# Autodesk Inventor assembly: Shooting Mechanism Assembly
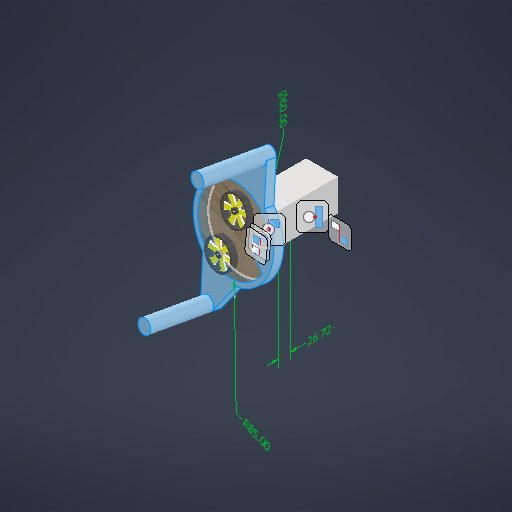
[picture p0: Inventor's stored thumbnail of the model, 512x512]
Saved by Autodesk Inventor 2026.2 (Build 302298000, 298)
## iProperties
Created: 2026-03-02
Part Number: Shooting Mechanism Assembly
Document SubType Name: Assembly
Designer: abdul
Author: abdul
## Documents named in this file (7)
- C:\Users\danda\OneDrive\Desktop\Basics Of Mecha\Project\Shooting Mechanism CAD\Shooting Mechanism Assembly.iam
- C:\Users\danda\OneDrive\Desktop\Basics Of Mecha\Project\Shooting Mechanism CAD\Base.ipt
- C:\Users\danda\OneDrive\Desktop\Basics Of Mecha\Project\Shooting Mechanism CAD\flywheel.ipt
- C:\Users\danda\OneDrive\Desktop\Basics Of Mecha\Project\Shooting Mechanism CAD\Dc Motor 3mm D Shaft.ipt
- C:\Users\danda\OneDrive\Desktop\Basics Of Mecha\Project\Ball Joint.iam
- C:\Users\danda\OneDrive\Desktop\Basics Of Mecha\Project\shootingstand.ipt
- C:\Users\danda\OneDrive\Desktop\Basics Of Mecha\Project\shooter handle.ipt
## Components (8 placed, 6 different names)
1. Base:1 — Mate:1, Mate:2, Mate:3, Mate:4, Mate:16, Mate:17, Flush:1, Mate:19, Mate:20
2. Dc Motor 3mm D Shaft:1 — Mate:1, Mate:4, Mate:9, Mate:11
3. Dc Motor 3mm D Shaft:2 — Mate:2, Mate:3, Mate:6, Mate:8, Mate:10
4. flywheel:2 — Mate:6, Mate:8, Mate:10
5. flywheel:3 — Mate:9, Mate:11
6. Ball Joint:1 [sub-assembly] — Mate:16, Mate:17, Mate:18, Tangent:1
7. shootingstand:1 — Mate:13, Mate:14, Mate:15, Mate:18, Tangent:1
8. shooter handle:1 — Flush:1, Mate:19, Mate:20
## Relationships (19: Mate 17, Tangent 1, Flush 1)
- Mate:1: Base:1 ↔ Dc Motor 3mm D Shaft:1
- Mate:2: Base:1 ↔ Dc Motor 3mm D Shaft:2
- Mate:3: Base:1 ↔ Dc Motor 3mm D Shaft:2
- Mate:4: Base:1 ↔ Dc Motor 3mm D Shaft:1
- Mate:6: Dc Motor 3mm D Shaft:2 ↔ flywheel:2
- Mate:8: Dc Motor 3mm D Shaft:2 ↔ flywheel:2
- Mate:9: Dc Motor 3mm D Shaft:1 ↔ flywheel:3
- Mate:10: Dc Motor 3mm D Shaft:2 ↔ flywheel:2
- Mate:11: Dc Motor 3mm D Shaft:1 ↔ flywheel:3
- Mate:13: shootingstand:1
- Mate:14: shootingstand:1
- Mate:15: shootingstand:1
- Mate:16: Base:1 ↔ Ball Joint:1
- Mate:17: Base:1 ↔ Ball Joint:1
- Mate:18: Ball Joint:1 ↔ shootingstand:1
- Tangent:1: Ball Joint:1 ↔ shootingstand:1
- Flush:1: Base:1 ↔ shooter handle:1
- Mate:19: Base:1 ↔ shooter handle:1
- Mate:20: Base:1 ↔ shooter handle:1
